# Autodesk Inventor assembly: Schaufelrad
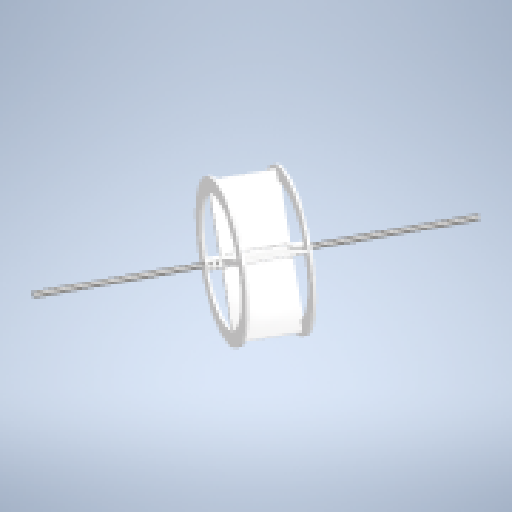
[picture p0: Inventor's stored thumbnail of the model, 512x512]
Saved by Autodesk Inventor 2024.4 (Build 284460000, 460)
## iProperties
Created: 2026-01-10
Part Number: Schaufelrad
Description: Schaufelrad
Document SubType Name: Assembly
Designer: Philf
Mass: 7926.27 g
Surface Area: 9708.09 cm^2
Volume: 3958.37 cm^3
Density: 2.00241 g/cm^3
Masse[kg]: 7,926 kg
## Documents named in this file (7)
- C:\Users\Philf\Documents\Vault\Daten\I60-Konstruktion\I60-Gruppe-7\schaufelrad\Schaufelrad.iam
- C:\Users\Philf\Documents\Vault\Daten\I60-Konstruktion\I60-Gruppe-7\schaufelrad\Seitenscheibe.ipt
- C:\Users\Philf\Documents\Vault\Daten\I60-Konstruktion\I60-Gruppe-7\schaufelrad\Schaufelplatten.ipt
- C:\Users\Philf\Documents\Vault\Daten\I60-Konstruktion\I60-Gruppe-7\schaufelrad\Distanz.ipt
- C:\Users\Philf\Documents\Vault\Daten\I60-Konstruktion\I60-Gruppe-7\schaufelrad\Stangeschaufelrad.ipt
- C:\Users\Philf\Documents\Vault\Daten\I60-Konstruktion\I60-Gruppe-7\Tritt\Stopper.ipt
- C:\Users\Philf\Documents\Vault\Normteile\de-DE\ISO 4762(1)\DIN EN ISO 4762 - M5 x 20.ipt
## Components (14 placed, 6 different names)
1. Seitenscheibe:1 — Passend:1, Passend:2, Fluchtend:1, Passend:3, Passend:4, Passend:5, Passend:6, Passend:7, Passend:8, Passend:12, Passend:13, Fluchtend:2, Passend:15, Passend:18
2. Seitenscheibe:2 — Passend:1, Passend:2, Fluchtend:1, Passend:9, Passend:10, Passend:11, Passend:14, Passend:16, Passend:20, Fluchtend:3
3. Schaufelplatten:1 — Passend:12, Passend:13, Passend:14
4. Schaufelplatten:2 — Passend:3, Passend:4, Passend:5
5. Schaufelplatten:3 — Passend:6, Passend:7, Passend:8
6. Schaufelplatten:4 — Passend:9, Passend:10, Passend:11
7. Distanz:1 — Fluchtend:2, Passend:15
8. Stangeschaufelrad:1 — Passend:16, Passend:17, Passend:19, Fluchtend:3
9. Stopper:1 — Passend:17, Passend:18, Winkel:1, Einfügen:3, Einfügen:4
10. Stopper:2 — Passend:19, Passend:20, Winkel:2, Einfügen:1, Einfügen:2
11. DIN EN ISO 4762 M5 x 20:1 — Einfügen:1
12. DIN EN ISO 4762 M5 x 20:2 — Einfügen:2
13. DIN EN ISO 4762 M5 x 20:3 — Einfügen:3
14. DIN EN ISO 4762 M5 x 20:4 — Einfügen:4
## Relationships (29: Mate 20, Insert 4, Flush 3, Angle 2)
- Passend:1 [Mate] (200 mm): Seitenscheibe:1 ↔ Seitenscheibe:2
- Passend:2 [Mate]: Seitenscheibe:1 ↔ Seitenscheibe:2
- Fluchtend:1 [Flush]: Seitenscheibe:1 ↔ Seitenscheibe:2
- Passend:3 [Mate]: Seitenscheibe:1 ↔ Schaufelplatten:2
- Passend:4 [Mate]: Seitenscheibe:1 ↔ Schaufelplatten:2
- Passend:5 [Mate]: Seitenscheibe:1 ↔ Schaufelplatten:2
- Passend:6 [Mate]: Seitenscheibe:1 ↔ Schaufelplatten:3
- Passend:7 [Mate]: Seitenscheibe:1 ↔ Schaufelplatten:3
- Passend:8 [Mate]: Seitenscheibe:1 ↔ Schaufelplatten:3
- Passend:9 [Mate]: Seitenscheibe:2 ↔ Schaufelplatten:4
- Passend:10 [Mate]: Seitenscheibe:2 ↔ Schaufelplatten:4
- Passend:11 [Mate]: Seitenscheibe:2 ↔ Schaufelplatten:4
- Passend:12 [Mate]: Seitenscheibe:1 ↔ Schaufelplatten:1
- Passend:13 [Mate]: Seitenscheibe:1 ↔ Schaufelplatten:1
- Passend:14 [Mate]: Seitenscheibe:2 ↔ Schaufelplatten:1
- Fluchtend:2 [Flush]: Seitenscheibe:1 ↔ Distanz:1
- Passend:15 [Mate]: Seitenscheibe:1 ↔ Distanz:1
- Passend:16 [Mate]: Seitenscheibe:2 ↔ Stangeschaufelrad:1
- Passend:17 [Mate]: Stangeschaufelrad:1 ↔ Stopper:1
- Passend:18 [Mate]: Seitenscheibe:1 ↔ Stopper:1
- Passend:19 [Mate]: Stangeschaufelrad:1 ↔ Stopper:2
- Passend:20 [Mate]: Seitenscheibe:2 ↔ Stopper:2
- Winkel:1 [Angle] (0 deg): Stopper:1
- Winkel:2 [Angle] (0 deg): Stopper:2
- Fluchtend:3 [Flush] (560 mm): Seitenscheibe:2 ↔ Stangeschaufelrad:1
- Einfügen:1 [Insert]: Stopper:2 ↔ DIN EN ISO 4762 M5 x 20:1
- Einfügen:2 [Insert]: Stopper:2 ↔ DIN EN ISO 4762 M5 x 20:2
- Einfügen:3 [Insert]: Stopper:1 ↔ DIN EN ISO 4762 M5 x 20:3
- Einfügen:4 [Insert]: Stopper:1 ↔ DIN EN ISO 4762 M5 x 20:4
